# Autodesk Inventor assembly: controladores
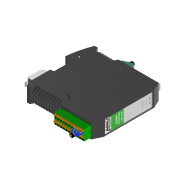
[picture p0: Inventor's stored thumbnail of the model, 180x180]
Saved by Autodesk Inventor 2022 (Build 260153000, 153)
## iProperties
Created: 2022-11-18
Part Number: controladores
Document SubType Name: Assembly
Designer: ferna
Author: ferna
## Documents named in this file (9)
- C:\Users\ferna\Documents\Bocas\Prototipo_09\amci\controladores.iam
- C:\Users\ferna\Documents\Bocas\Prototipo_09\amci\controlador.ipt
- C:\Users\ferna\Downloads\rj-jack-1.snapshot.2\RJ45 Jack.iam
- C:\Users\ferna\Downloads\pluggable-terminal-connector-2-pin-1.snapshot.1\Terminal Connector.iam
- C:\Users\ferna\Documents\Bocas\Prototipo_09\amci\conectores.ipt
- C:\Users\ferna\Documents\Bocas\Prototipo_09\amci\conectores_macho.ipt
- C:\Users\ferna\Downloads\rj45-ethernet-plug\Part29.ipt
- C:\Users\ferna\Documents\Bocas\Prototipo_09\amci\conector_motores.ipt
- C:\Users\ferna\Documents\Bocas\Prototipo_09\amci\controladores\AIP\Cable and Harness\controladores.Harness1.iam
## Components (12 placed, 8 different names)
1. controlador:1 — Mate:1, Mate:2, Mate:3, Mate:4, Mate:5, Mate:6, Flush:1, Mate:7, Mate:8, Flush:2, Mate:10, Mate:11, Mate:12
2. RJ45 Jack:1 [sub-assembly] — Mate:1, Mate:2, Mate:3, Mate:16, Mate:19, Mate:20, Mate:21
3. RJ45 Jack:2 [sub-assembly] — Mate:4, Mate:5, Mate:6, Mate:17, Mate:18
4. Terminal Connector:1 [sub-assembly] — Flush:2, Mate:9, Flush:3, Mate:22, Tangent:1, Tangent:2
5. Terminal Connector:2 [sub-assembly] — Flush:1, Mate:7, Mate:8, Mate:9, Flush:3
6. conectores:1 — Mate:10, Mate:11, Mate:12, Mate:13, Mate:14, Mate:15
7. conectores_macho:1 — Mate:13, Mate:14, Mate:15, Mate:23, Tangent:3, Tangent:4
8. Part29:1 — Mate:16, Mate:17, Mate:18
9. Part29:2 — Mate:19, Mate:20, Mate:21
10. conector_motores:1 — Mate:22, Tangent:1, Tangent:2
11. Harness1 [sub-assembly]
12. conector_motores:2 — Mate:23, Tangent:3, Tangent:4
## Relationships (30: Mate 23, Tangent 4, Flush 3)
- Mate:1: controlador:1 ↔ RJ45 Jack:1
- Mate:2: controlador:1 ↔ RJ45 Jack:1
- Mate:3: controlador:1 ↔ RJ45 Jack:1
- Mate:4: controlador:1 ↔ RJ45 Jack:2
- Mate:5: controlador:1 ↔ RJ45 Jack:2
- Mate:6: controlador:1 ↔ RJ45 Jack:2
- Flush:1 (-10 mm): controlador:1 ↔ Terminal Connector:2
- Mate:7: controlador:1 ↔ Terminal Connector:2
- Mate:8: controlador:1 ↔ Terminal Connector:2
- Flush:2 (-10 mm): controlador:1 ↔ Terminal Connector:1
- Mate:9: Terminal Connector:1 ↔ Terminal Connector:2
- Flush:3: Terminal Connector:1 ↔ Terminal Connector:2
- Mate:10: controlador:1 ↔ conectores:1
- Mate:11: controlador:1 ↔ conectores:1
- Mate:12: controlador:1 ↔ conectores:1
- Mate:13 (0.5 mm): conectores:1 ↔ conectores_macho:1
- Mate:14: conectores:1 ↔ conectores_macho:1
- Mate:15: conectores:1 ↔ conectores_macho:1
- Mate:16: RJ45 Jack:1 ↔ Part29:1
- Mate:17: RJ45 Jack:2 ↔ Part29:1
- Mate:18: RJ45 Jack:2 ↔ Part29:1
- Mate:19: RJ45 Jack:1 ↔ Part29:2
- Mate:20: RJ45 Jack:1 ↔ Part29:2
- Mate:21: RJ45 Jack:1 ↔ Part29:2
- Mate:22 (10 mm): Terminal Connector:1 ↔ conector_motores:1
- Tangent:1 (8.5 mm): Terminal Connector:1 ↔ conector_motores:1
- Tangent:2 (-10 mm): Terminal Connector:1 ↔ conector_motores:1
- Mate:23 (10 mm): conectores_macho:1 ↔ conector_motores:2
- Tangent:3: conectores_macho:1 ↔ conector_motores:2
- Tangent:4: conectores_macho:1 ↔ conector_motores:2
